# Autodesk Inventor assembly: CLB_076_ScissorMidBarrAssembly
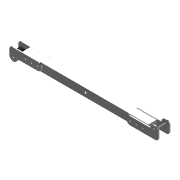
[picture p0: Inventor's stored thumbnail of the model, 180x180]
Saved by Autodesk Inventor 2018 (Build 220112000, 112)
## iProperties
Created: 2020-02-13
Part Number: CLB_076_ScissorMidBarrAssembly
Document SubType Name: Assembly
Designer: Cooper
Author: Cooper
## Documents named in this file (9)
- C:\Users\Myers.000\Documents\GrabCAD\Infinite Recharge 2020\Build season\CLB_076_ScissorMidBarrAssembly.iam
- C:\Users\Myers.000\Documents\GrabCAD\Infinite Recharge 2020\Build season\CLB_027_LifterBracket.ipt
- C:\Users\Myers.000\Documents\GrabCAD\Infinite Recharge 2020\Build season\CLB_040_ScissorLiftSpacer2.ipt
- C:\Users\Myers.000\Documents\GrabCAD\Infinite Recharge 2020\Build season\CLB_046_ClevisPinScissors.ipt
- C:\Users\Myers.000\Documents\GrabCAD\Infinite Recharge 2020\Build season\CLB_052_ScissorLiftPlug.ipt
- C:\Users\Myers.000\Documents\GrabCAD\Infinite Recharge 2020\Build season\CLB_049_MiddleBarFourPartScissors.ipt
- C:\Users\Myers.000\Documents\GrabCAD\Infinite Recharge 2020\Build season\CLB_047_SpringSpacer.ipt
- C:\Users\Myers.000\Documents\GrabCAD\Infinite Recharge 2020\Build season\CLB_045_TorsionSpring_MM_9271K129.ipt
- CLB_027_LifterBracket.ipt
## Components (12 placed, 7 different names)
1. CLB_049_MiddleBarFourPartScissors:2 — Mate:14, Flush:24, Mate:15, Flush:26, Flush:27, Mate:17, Mate:18, Mate:36, Mate:37, Flush:46, Mate:38, Flush:47, Mate:41, Flush:48, Flush:49, Mate:42, Flush:54, Flush:56, Mate:44, Mate:45, Flush:59, Flush:60
2. CLB_027_LifterBracket:6 — Mate:15, Flush:26, Flush:27, Flush:53, Flush:58
3. CLB_027_LifterBracket:7 — Mate:14, Flush:24, Flush:53, Insert:2
4. CLB_027_LifterBracket:11 — Mate:20, Insert:1, Flush:49, Flush:52, Mate:42
5. CLB_027_LifterBracket:12 — Mate:19, Flush:48, Flush:52
6. CLB_040_ScissorLiftSpacer2:5 — Mate:18, Mate:20, Flush:56, Flush:60
7. CLB_040_ScissorLiftSpacer2:6 — Mate:17, Mate:19, Flush:54, Flush:59
8. CLB_046_ClevisPinScissors:3 — Insert:1
9. CLB_052_ScissorLiftPlug:1 — Mate:36, Mate:37, Flush:46, Mate:38
10. CLB_052_ScissorLiftPlug:3 — Flush:47, Mate:44, Mate:45
11. CLB_047_SpringSpacer:1 — Insert:2, Mate:43
12. CLB_045_TorsionSpring_MM_9271K129:1 — Mate:43, Flush:58
## Relationships (30: Mate 14, Flush 14, Insert 2)
- Mate:14: CLB_049_MiddleBarFourPartScissors:2 ↔ CLB_027_LifterBracket:7
- Flush:24: CLB_049_MiddleBarFourPartScissors:2 ↔ CLB_027_LifterBracket:7
- Mate:15: CLB_049_MiddleBarFourPartScissors:2 ↔ CLB_027_LifterBracket:6
- Flush:26: CLB_049_MiddleBarFourPartScissors:2 ↔ CLB_027_LifterBracket:6
- Flush:27 (-38.1 mm): CLB_049_MiddleBarFourPartScissors:2 ↔ CLB_027_LifterBracket:6
- Mate:17: CLB_049_MiddleBarFourPartScissors:2 ↔ CLB_040_ScissorLiftSpacer2:6
- Mate:18: CLB_049_MiddleBarFourPartScissors:2 ↔ CLB_040_ScissorLiftSpacer2:5
- Mate:19: CLB_027_LifterBracket:12 ↔ CLB_040_ScissorLiftSpacer2:6
- Mate:20: CLB_027_LifterBracket:11 ↔ CLB_040_ScissorLiftSpacer2:5
- Insert:1: CLB_027_LifterBracket:11 ↔ CLB_046_ClevisPinScissors:3
- Mate:36: CLB_049_MiddleBarFourPartScissors:2 ↔ CLB_052_ScissorLiftPlug:1
- Mate:37: CLB_049_MiddleBarFourPartScissors:2 ↔ CLB_052_ScissorLiftPlug:1
- Flush:46: CLB_049_MiddleBarFourPartScissors:2 ↔ CLB_052_ScissorLiftPlug:1
- Mate:38: CLB_049_MiddleBarFourPartScissors:2 ↔ CLB_052_ScissorLiftPlug:1
- Flush:47: CLB_049_MiddleBarFourPartScissors:2 ↔ CLB_052_ScissorLiftPlug:3
- Mate:41: CLB_049_MiddleBarFourPartScissors:2
- Flush:48: CLB_049_MiddleBarFourPartScissors:2 ↔ CLB_027_LifterBracket:12
- Flush:49: CLB_049_MiddleBarFourPartScissors:2 ↔ CLB_027_LifterBracket:11
- Flush:52: CLB_027_LifterBracket:11 ↔ CLB_027_LifterBracket:12
- Mate:42: CLB_049_MiddleBarFourPartScissors:2 ↔ CLB_027_LifterBracket:11
- Flush:53: CLB_027_LifterBracket:6 ↔ CLB_027_LifterBracket:7
- Flush:54: CLB_049_MiddleBarFourPartScissors:2 ↔ CLB_040_ScissorLiftSpacer2:6
- Flush:56: CLB_049_MiddleBarFourPartScissors:2 ↔ CLB_040_ScissorLiftSpacer2:5
- Insert:2: CLB_027_LifterBracket:7 ↔ CLB_047_SpringSpacer:1
- Mate:43: CLB_047_SpringSpacer:1 ↔ CLB_045_TorsionSpring_MM_9271K129:1
- Flush:58 (-2.54 mm): CLB_027_LifterBracket:6 ↔ CLB_045_TorsionSpring_MM_9271K129:1
- Mate:44: CLB_049_MiddleBarFourPartScissors:2 ↔ CLB_052_ScissorLiftPlug:3
- Mate:45: CLB_049_MiddleBarFourPartScissors:2 ↔ CLB_052_ScissorLiftPlug:3
- Flush:59: CLB_049_MiddleBarFourPartScissors:2 ↔ CLB_040_ScissorLiftSpacer2:6
- Flush:60: CLB_049_MiddleBarFourPartScissors:2 ↔ CLB_040_ScissorLiftSpacer2:5
